# Autodesk Inventor assembly: Assembly_Cube_Flashlight_v3
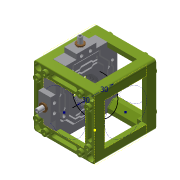
[picture p0: Inventor's stored thumbnail of the model, 180x180]
Saved by Autodesk Inventor 2019.4 (Build 234330000, 330)
## iProperties
Created: 2020-12-04
Part Number: Assembly_Cube_Flashlight_v3
Document SubType Name: Assembly
Designer: UC2
Author: UC2
## Documents named in this file (5)
- C:\Users\diederichbenedict\Dropbox\Dokumente\Promotion\PROJECTS\UC2\02_CAD\INVENTOR\uc2_v3\Assembly_Cube_Flexuremanipulator_v3.iam
- C:\Users\diederichbenedict\Dropbox\Dokumente\Promotion\PROJECTS\UC2\02_CAD\INVENTOR\uc2_v3\Assembly_Cube_empty_IM_v3.iam
- C:\Users\diederichbenedict\Dropbox\Dokumente\Promotion\PROJECTS\UC2\02_CAD\INVENTOR\uc2_v3\20_Cube_Inser_Flexuremanipulator_v3.ipt
- C:\Users\diederichbenedict\Downloads\00_F6SSN2P-Step.ipt
- C:\Users\diederichbenedict\Downloads\00_F6SS088-Step.ipt
## Components (6 placed, 4 different names)
1. Assembly_Cube_empty_IM_v3:1 [sub-assembly] — Flush:3, Flush:4
2. 20_Cube_Inser_Flexuremanipulator_v3:1 — Flush:3, Flush:4, Insert:1, Insert:4
3. 00_F6SSN2P-Step:1 — Insert:1, Insert:2
4. 00_F6SS088-Step:1 — Insert:2
5. 00_F6SSN2P-Step:2 — Insert:4
6. 00_F6SS088-Step:2
## Relationships (6: Insert 4, Flush 2)
- Flush:3: Assembly_Cube_empty_IM_v3:1 ↔ 20_Cube_Inser_Flexuremanipulator_v3:1
- Flush:4: Assembly_Cube_empty_IM_v3:1 ↔ 20_Cube_Inser_Flexuremanipulator_v3:1
- Insert:1: 20_Cube_Inser_Flexuremanipulator_v3:1 ↔ 00_F6SSN2P-Step:1
- Insert:2 (-5 mm): 00_F6SSN2P-Step:1 ↔ 00_F6SS088-Step:1
- [Insert] (-5 mm): 00_F6SSN2P-Step:2 ↔ 00_F6SS088-Step:2
- Insert:4: 20_Cube_Inser_Flexuremanipulator_v3:1 ↔ 00_F6SSN2P-Step:2
## Named parameters: d14_d13 = -5 mm
